# Autodesk Inventor assembly: E-NTBGT13-8
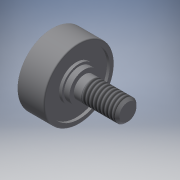
[picture p0: Inventor's stored thumbnail of the model, 180x180]
Saved by Autodesk Inventor 2019 (Build 230136000, 136)
## iProperties
Category: PARTsolutions
Company: MISUMI
Created: 2024-10-07
Part Number: E-NTBGT13-8
Catalog Web Link: www.cadenas.de
Description: E-NTBGT, E-NTSBGT-Economy Bearings with Male Threads Long Type
Vendor: MISUMI
Document SubType Name: Assembly
Designer: psAdmin
Manufacturer: MISUMI
Mass: 0.707064 g
Surface Area: 7.89012 cm^2
Volume: 0.707064 cm^3
Density: 1 g/cm^3
Title: E-NTBGT13-8
Author: Cadenas PARTsolutions
Comments: Economy Bearings with Male Threads Long Type
PSOL_IDENT_0: {$CADENAS_DATA/23d-libs/misumi/metric/53_rollers/e_ntsbgt_asmtab.prj},191 {VTYP=3D},{STYP=ASSTAB},{N
PSOL_IDENT_1: B=E-NTBGT13-8},{LINA=E-NTBGT13-8},{NN=E-NTBGT, E-NTSBGT},{DATE=17.05.2024 10:15:32},{GEOMDATE=17.05.
PSOL_IDENT_2: 2024 10:04:59},{VERSION=},{LINEID=30},{WBVAR=MATB},{WBNUMERIC=}  {NB=E-NTBGT13-8},{LINA=E-NTBGT13-8}
PSOL_IDENT_3: ,{KT=DUMMY},{PN=E-NTBGT13-8},{TYPE=E-NTBGT},{TS=T},{TSALG= '','Standard Male Thread','T','Long Male
PSOL_IDENT_4: Thread' },{MATB=},{MATBALG= '','Steel','S','Stainless Steel' },{MATS=Stainless Steel},{ST=Electroles
PSOL_IDENT_5: s Nickel Plating},{D=13},{L=8},{B=5.0},{DD=4},{AA=1.0},{G=2.0},{M=M4},{M1=4},{BE=624ZZ},{LSM=5},{LLM=
PSOL_IDENT_6: 8},{D1=5.6},{B1=4.8000},{G1=1.5},{DIA=0.400},{PITCH=0.7},{Z=0.2},{PPATH=e_ntsbgt/e_ntsbgt_asmtpl.prj
PSOL_IDENT_7: }
NB: E-NTBGT13-8
NN: E-NTBGT, E-NTSBGT
NT: Economy Bearings with Male Threads Long Type
NBSYN: $PN.
LINA: E-NTBGT13-8
CATALOG: Misumi
PN: E-NTBGT13-8
MATB: Steel
D: 13
L: 8
B: 5
DD: 4
AA: 1
G: 2
M: M4
BE: 624ZZ
SUPPLIER: MISUMI
ARTICLENO: E-NTBGT13-8
BOMINFO: E-NTBGT13-8
CREATOR: CADENAS GmbH
## Documents named in this file (3)
- e:\temp\worker_COMMON_460\temp\tmp_8032_104_KeLCd\format_0\E-NTBGT13-8.iam
- e:\temp\worker_COMMON_460\temp\tmp_8032_104_KeLCd\format_0\E-NTBGT13-8_b.ipt
- e:\temp\worker_COMMON_460\temp\tmp_8032_104_KeLCd\format_0\B624ZZ.ipt
## Components (2 placed, 2 different names)
1. E-NTBGT13-8_b:1 — shaft_to_bearing_XY@1 <-> to_housing_XY@2, shaft_to_bearing_Z@1 <-> to_housing_Z@2, shaft_to_bearing_YZ@1 <-> to_housing_YZ@2
2. B624ZZ:1 — shaft_to_bearing_XY@1 <-> to_housing_XY@2, shaft_to_bearing_Z@1 <-> to_housing_Z@2, shaft_to_bearing_YZ@1 <-> to_housing_YZ@2
## Relationships (3: Mate 2, Angle 1)
- shaft_to_bearing_XY@1 <-> to_housing_XY@2 [Mate]: E-NTBGT13-8_b:1 ↔ B624ZZ:1
- shaft_to_bearing_Z@1 <-> to_housing_Z@2 [Mate]: E-NTBGT13-8_b:1 ↔ B624ZZ:1
- shaft_to_bearing_YZ@1 <-> to_housing_YZ@2 [Angle] (0 deg): E-NTBGT13-8_b:1 ↔ B624ZZ:1
